# Autodesk Inventor assembly: Housing_Assembly_2_0_2
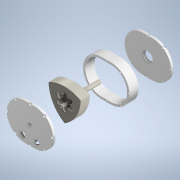
[picture p0: Inventor's stored thumbnail of the model, 180x180]
Saved by Autodesk Inventor 2021 (Build 250183000, 183)
## iProperties
Created: 2021-04-19
Part Number: Housing_Assembly_2_0_2
Document SubType Name: Assembly
Designer: lucia
Author: lucia
## Documents named in this file (7)
- E:\Documents\Inventor\Fixed Rotor Wankel Engine\Assemblies\Housing_Assembly_2_0_2.iam
- E:\Documents\Inventor\Fixed Rotor Wankel Engine\Parts\Rotor_Mount.ipt
- E:\Documents\Inventor\Fixed Rotor Wankel Engine\Parts\Eccentric_Shaft_2.ipt
- E:\Documents\Inventor\Fixed Rotor Wankel Engine\Parts\Rotor_Geared_6t_Mountable.ipt
- E:\Documents\Inventor\Fixed Rotor Wankel Engine\Parts\Side_Plate_Combined_Intake_Exhaust.ipt
- E:\Documents\Inventor\Fixed Rotor Wankel Engine\Parts\Housing.ipt
- E:\Documents\Inventor\Fixed Rotor Wankel Engine\Parts\Side_Plate_Blank.ipt
## Components (6 placed, 6 different names)
1. Rotor_Mount:1 — Mate:1, Mate:2, Mate:3, Mate:4
2. Eccentric_Shaft_2:1 — Mate:3, Mate:4, Mate:5, Mate:6, Mate:8
3. Rotor_Geared_6t_Mountable:1 — Mate:5, Mate:6, Mate:7
4. Side_Plate_Combined_Intake_Exhaust:1 — Mate:7, Mate:8, Mate:9, Mate:10, Mate:11
5. Housing:1 — Mate:9, Mate:10, Mate:11, Mate:12, Mate:13, Mate:14
6. Side_Plate_Blank:1 — Mate:12, Mate:13, Mate:14
## Relationships (14: Mate 14)
- Mate:1: Rotor_Mount:1
- Mate:2: Rotor_Mount:1
- Mate:3: Rotor_Mount:1 ↔ Eccentric_Shaft_2:1
- Mate:4: Rotor_Mount:1 ↔ Eccentric_Shaft_2:1
- Mate:5: Eccentric_Shaft_2:1 ↔ Rotor_Geared_6t_Mountable:1
- Mate:6: Eccentric_Shaft_2:1 ↔ Rotor_Geared_6t_Mountable:1
- Mate:7 (177.8 mm): Rotor_Geared_6t_Mountable:1 ↔ Side_Plate_Combined_Intake_Exhaust:1
- Mate:8: Eccentric_Shaft_2:1 ↔ Side_Plate_Combined_Intake_Exhaust:1
- Mate:9 (406.4 mm): Side_Plate_Combined_Intake_Exhaust:1 ↔ Housing:1
- Mate:10: Side_Plate_Combined_Intake_Exhaust:1 ↔ Housing:1
- Mate:11: Side_Plate_Combined_Intake_Exhaust:1 ↔ Housing:1
- Mate:12 (177.8 mm): Housing:1 ↔ Side_Plate_Blank:1
- Mate:13: Housing:1 ↔ Side_Plate_Blank:1
- Mate:14: Housing:1 ↔ Side_Plate_Blank:1
